# Autodesk Inventor assembly: Backplane
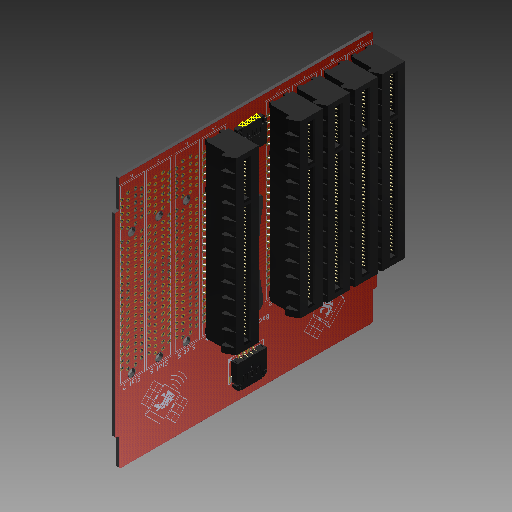
[picture p0: Inventor's stored thumbnail of the model, 512x512]
Saved by Autodesk Inventor 2018 (Build 220112000, 112)
## iProperties
Created: 2018-10-18
Part Number: Backplane
Document SubType Name: Assembly
Designer: Bradley
Author: Bradley
## Documents named in this file (7)
- C:\Users\Bradley\Documents\GitHub\CougSat1-Hardware\CougSat1-Backplane\CADModel\Native\Backplane.iam
- C:\Users\Bradley\Documents\GitHub\CougSat1-Hardware\CougSat1-Backplane\CADModel\Native\Backplane_PCB.ipt
- C:\Users\Bradley\Documents\GitHub\CougSat1-Hardware\CougSat1-Backplane\CADModel\Native\Backplane_CenterNut.ipt
- C:\Users\Bradley\Documents\GitHub\Resources\SupplierDocuments\04 - Connectors SMT\04-0001\04-0001.iam
- C:\Users\Bradley\Documents\GitHub\Resources\SupplierDocuments\05 - Connectors THT\05-0006\05-0006.ipt
- C:\Users\Bradley\Documents\GitHub\Resources\SupplierDocuments\11 - Capacitor Ceramic 1608\11-104A\11-104A.ipt
- C:\Users\Bradley\Documents\GitHub\Resources\SupplierDocuments\21 - Resistor 1608\21-0000\21-0000.ipt
## Components (13 placed, 6 different names)
1. 04-0001:1 [sub-assembly] — Mate:5, Flush:3, Mate:7
2. 04-0001:2 [sub-assembly] — Mate:6, Mate:8, Flush:4
3. 05-0006:1 — Mate:21, Mate:30, Angle:1
4. 05-0006:2 — Mate:22, Mate:29, Angle:2
5. 05-0006:3 — Mate:23, Mate:28, Angle:3
6. 05-0006:4 — Mate:24, Mate:27, Angle:4
7. 05-0006:5 — Mate:25, Mate:26, Angle:5
8. 11-104A:1 — Mate:11, Mate:13, Mate:14
9. 11-104A:2 — Mate:12, Mate:17, Mate:18
10. 21-0000:1 — Mate:9, Flush:17
11. 21-0000:2 — Mate:10, Flush:21
12. Backplane_CenterNut:1 — Insert:17, Insert:18
13. Backplane_PCB:1 — Mate:5, Mate:6, Mate:9, Mate:10, Mate:11, Mate:12, Insert:17, Insert:18, Mate:21, Mate:22, Mate:23, Mate:24, Mate:25, Mate:26, Mate:27, Mate:28, Mate:29, Mate:30
## Relationships (35: Mate 24, Angle 5, Flush 4, Insert 2)
- Mate:5: 04-0001:1 ↔ Backplane_PCB:1
- Mate:6: 04-0001:2 ↔ Backplane_PCB:1
- Flush:3: 04-0001:1
- Mate:7 (-29 mm): 04-0001:1
- Mate:8: 04-0001:2
- Flush:4 (29 mm): 04-0001:2
- Mate:9: 21-0000:1 ↔ Backplane_PCB:1
- Mate:10: 21-0000:2 ↔ Backplane_PCB:1
- Mate:11: 11-104A:1 ↔ Backplane_PCB:1
- Mate:12: 11-104A:2 ↔ Backplane_PCB:1
- Mate:13 (-1.8 mm): 11-104A:1
- Mate:14 (-9.5 mm): 11-104A:1
- [Mate] (1.8 mm): 21-0000:1
- Flush:17 (-9.5 mm): 21-0000:1
- Insert:17: Backplane_CenterNut:1 ↔ Backplane_PCB:1
- Insert:18: Backplane_CenterNut:1 ↔ Backplane_PCB:1
- Mate:17 (-1.8 mm): 11-104A:2
- Mate:18 (9.5 mm): 11-104A:2
- [Mate] (1.8 mm): 21-0000:2
- Flush:21 (9.5 mm): 21-0000:2
- Mate:21: 05-0006:1 ↔ Backplane_PCB:1
- Mate:22: 05-0006:2 ↔ Backplane_PCB:1
- Mate:23: 05-0006:3 ↔ Backplane_PCB:1
- Mate:24: 05-0006:4 ↔ Backplane_PCB:1
- Mate:25: 05-0006:5 ↔ Backplane_PCB:1
- Mate:26: 05-0006:5 ↔ Backplane_PCB:1
- Mate:27: 05-0006:4 ↔ Backplane_PCB:1
- Mate:28: 05-0006:3 ↔ Backplane_PCB:1
- Mate:29: 05-0006:2 ↔ Backplane_PCB:1
- Mate:30: 05-0006:1 ↔ Backplane_PCB:1
- Angle:1 (0 deg): 05-0006:1
- Angle:2 (0 deg): 05-0006:2
- Angle:3 (0 deg): 05-0006:3
- Angle:4 (0 deg): 05-0006:4
- Angle:5 (0 deg): 05-0006:5
